# Autodesk Inventor assembly: White King
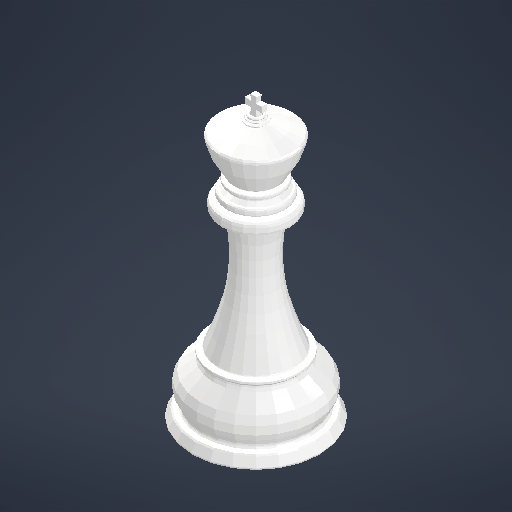
[picture p0: Inventor's stored thumbnail of the model, 512x512]
Saved by Autodesk Inventor 2026 (Build 300175000, 175)
## iProperties
Created: 2025-04-17
Part Number: White King
Document SubType Name: Assembly
Designer: ckyiu
Author: ckyiu
## Documents named in this file (4)
- F:\Chessboard-Design\Design\Core\Chess Pieces\White King.iam
- F:\Chessboard-Design\Design\Core\Chess Pieces\Parts\White King Body.ipt
- F:\Chessboard-Design\Design\Core\Chess Pieces\Parts\White King Head.ipt
- F:\Chessboard-Design\Design\Hardware\(9.5mm diameter 1.6mm height) 5862K143_Neodymium Magnet.ipt
## Components (3 placed, 3 different names)
1. White King Body:1 — Mate:1, Mate:2, Mate:3, Insert:1
2. White King Head:1 — Mate:1, Mate:2, Mate:3
3. (9.5mm diameter 1.6mm height) 5862K143_Neodymium Magnet:1 — Insert:1
## Relationships (4: Mate 3, Insert 1)
- Mate:1 (0.2 mm): White King Body:1 ↔ White King Head:1
- Mate:2 (0.2 mm): White King Body:1 ↔ White King Head:1
- Mate:3 (0.2 mm): White King Body:1 ↔ White King Head:1
- Insert:1: White King Body:1 ↔ (9.5mm diameter 1.6mm height) 5862K143_Neodymium Magnet:1
